# Autodesk Inventor assembly: ASY APN FDS way1
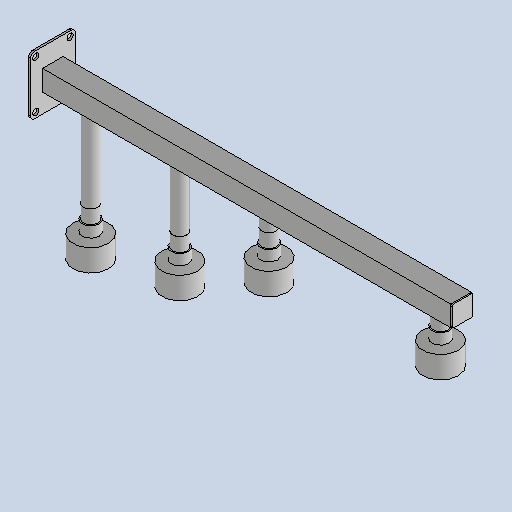
[picture p0: Inventor's stored thumbnail of the model, 512x512]
Saved by Autodesk Inventor 2025.1 (Build 291241020, 241B)
## iProperties
Created: 2025-07-02
Part Number: ASY APN FDS way1
Document SubType Name: Assembly
Designer: user
Author: user
## Documents named in this file (9)
- C:\Users\admin\Yandex.Disk\home pc\Inventor\ANP-Antipayuta\ASY APN FDS way1.iam
- C:\Users\admin\Yandex.Disk\home pc\Inventor\ANP-Antipayuta\APN 754 FDS 1200 way tube 1.ipt
- C:\Users\admin\Yandex.Disk\home pc\Inventor\ANP-Antipayuta\APN dummy filter element.ipt
- C:\Users\admin\Yandex.Disk\home pc\Inventor\ANP-Antipayuta\APN dummy pipe nippel.ipt
- C:\Users\admin\Yandex.Disk\home pc\Inventor\ANP-Antipayuta\APN 757 FDS 1200 way tube 4.ipt
- C:\Users\admin\Yandex.Disk\home pc\Inventor\ANP-Antipayuta\APN 1756 FDS 1200 way tube 6.ipt
- C:\Users\admin\Yandex.Disk\home pc\Inventor\ANP-Antipayuta\APN 1757 FDS 1200 way tube 7.ipt
- C:\Users\admin\Yandex.Disk\home pc\Inventor\ANP-Antipayuta\APN 760 FDS 1200 FLANGE 3.ipt
- C:\Users\admin\Yandex.Disk\home pc\Inventor\ANP-Antipayuta\APN 766 FDS 1200 CUP 1.ipt
## Components (14 placed, 8 different names)
1. PNS 754 FDS 1200 way tube 1.ipt:1 — Rigid:13
2. PNS dummy filter element.ipt:1
3. PNS dummy pipe nippel.ipt:1
4. PNS 757 FDS 1200 way tube 4.ipt:1
5. PNS dummy filter element.ipt:2
6. PNS dummy pipe nippel.ipt:2
7. PNS 758 FDS 1200 way tube 6.ipt:1
8. PNS dummy filter element.ipt:3
9. PNS dummy pipe nippel.ipt:3
10. PNS 759 FDS 1200 way tube 7.ipt:1
11. PNS dummy filter element.ipt:4
12. PNS dummy pipe nippel.ipt:4
13. PNS 760 FDS 1200 FLANGE 3.ipt:1
14. PNS 766 FDS 1200 CUP 1.ipt:1 — Rigid:13
## Relationships (13: WeldJoint 13)
- [WeldJoint]: PNS dummy filter element.ipt:1 ↔ PNS dummy pipe nippel.ipt:1
- [WeldJoint]: PNS 754 FDS 1200 way tube 1.ipt:1 ↔ PNS dummy pipe nippel.ipt:1
- [WeldJoint]: PNS dummy filter element.ipt:2 ↔ PNS dummy pipe nippel.ipt:2
- [WeldJoint]: PNS 757 FDS 1200 way tube 4.ipt:1 ↔ PNS dummy pipe nippel.ipt:2
- [WeldJoint]: PNS 754 FDS 1200 way tube 1.ipt:1 ↔ PNS 757 FDS 1200 way tube 4.ipt:1
- [WeldJoint]: PNS dummy filter element.ipt:3 ↔ PNS dummy pipe nippel.ipt:3
- [WeldJoint]: PNS 758 FDS 1200 way tube 6.ipt:1 ↔ PNS dummy pipe nippel.ipt:3
- [WeldJoint]: PNS dummy filter element.ipt:4 ↔ PNS dummy pipe nippel.ipt:4
- [WeldJoint]: PNS 759 FDS 1200 way tube 7.ipt:1 ↔ PNS dummy pipe nippel.ipt:4
- [WeldJoint]: PNS 754 FDS 1200 way tube 1.ipt:1 ↔ PNS 758 FDS 1200 way tube 6.ipt:1
- [WeldJoint]: PNS 754 FDS 1200 way tube 1.ipt:1 ↔ PNS 759 FDS 1200 way tube 7.ipt:1
- [WeldJoint] (-2 mm): PNS 754 FDS 1200 way tube 1.ipt:1 ↔ PNS 760 FDS 1200 FLANGE 3.ipt:1
- Rigid:13 [WeldJoint]: PNS 754 FDS 1200 way tube 1.ipt:1 ↔ PNS 766 FDS 1200 CUP 1.ipt:1
## Named parameters: d33_d31 = 0 mm, d37_d34_d31 = 0 mm, d43_d40_d37_d34_d31 = 0 mm, d44_d41 = 0 mm, d47_d45_d43_d40_d37_d34_d31 = 0 mm, d48_d46 = 0 mm
